# Autodesk Inventor assembly: aio_radiator_part
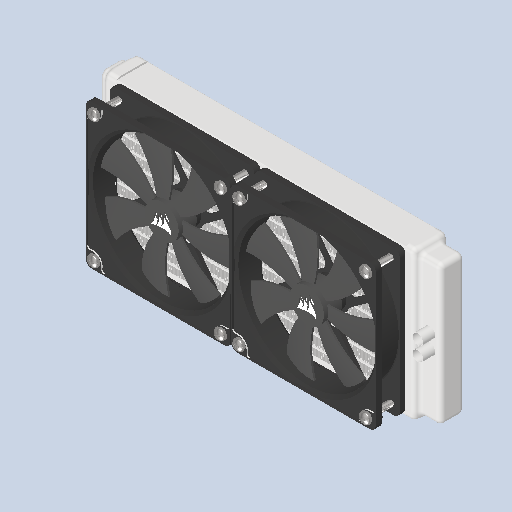
[picture p0: Inventor's stored thumbnail of the model, 512x512]
Saved by Autodesk Inventor 2022 (Build 260153000, 153)
## iProperties
Created: 2021-05-19
Part Number: aio_radiator_part
Document SubType Name: Assembly
Designer: 6128059
Author: 6128059
## Documents named in this file (9)
- C:\Users\sbbgi\Documents\GitHub\eatx_case\atx\resources\aio-cooler-1.snapshot.2\AIO Cooler\aio_radiator_part.iam
- C:\Users\sbbgi\Documents\GitHub\eatx_case\atx\resources\aio-cooler-1.snapshot.2\AIO Cooler\Kølerør.ipt
- C:\Users\sbbgi\Documents\GitHub\eatx_case\atx\resources\aio-cooler-1.snapshot.2\AIO Cooler\Gitter.ipt
- C:\Users\sbbgi\Documents\GitHub\eatx_case\atx\resources\aio-cooler-1.snapshot.2\AIO Cooler\Yderskal - Sheet metal.ipt
- C:\Users\sbbgi\Documents\GitHub\eatx_case\atx\resources\aio-cooler-1.snapshot.2\AIO Cooler\Radiator - Lukket ende.ipt
- C:\Users\sbbgi\Documents\GitHub\eatx_case\atx\resources\aio-cooler-1.snapshot.2\AIO Cooler\Radiator - Åben ende.ipt
- C:\Users\sbbgi\Documents\GitHub\eatx_case\atx\resources\aio-cooler-1.snapshot.2\AIO Cooler\120 mm fan assembly.iam
- C:\Users\sbbgi\Documents\GitHub\eatx_case\atx\resources\aio-cooler-1.snapshot.2\AIO Cooler\Rørende.ipt
- C:\Users\sbbgi\Documents\GitHub\eatx_case\atx\resources\aio-cooler-1.snapshot.2\AIO Cooler\ANSI B18.6.7M - M5x0,8 x 30(5).ipt
## Components (30 placed, 8 different names)
1. Kølerør:1 — Tangent:1, Mate:1, Tangent:2, Flush:1, Mate:11, Mate:12, Flush:2, Mate:13, Flush:3, Flush:4, Mate:14
2. Yderskal - Sheet metal:1 — Mate:8, Mate:9, Mate:10, Mate:11
3. Yderskal - Sheet metal:2 — Mate:2, Mate:3, Mate:4, Mate:5, Mate:6, Mate:7, Mate:12, Flush:2
4. 120 mm fan assembly:1 [sub-assembly] — Mate:2, Mate:3, Mate:4, Mate:10, Mate:32, Mate:33
5. 120 mm fan assembly:2 [sub-assembly] — Mate:5, Mate:6, Mate:7, Mate:8, Mate:9, Mate:30, Mate:31
6. Radiator - Åben ende:1 — Mate:13, Flush:3, Flush:4, Mate:15, Mate:16, Mate:20, Mate:21, Mate:22, Mate:23
7. Radiator - Lukket ende:1 — Mate:14, Mate:15, Mate:16
8. Rørende:3 — Mate:21, Mate:22
9. Rørende:4 — Mate:20, Mate:23
10. Gitter:1 — Tangent:1, Mate:1, Tangent:2, Flush:1
11. Gitter:2
12. Gitter:3
13. Gitter:4
14. Gitter:5
15. Gitter:6
16. Gitter:7
17. Gitter:8
18. Gitter:9
19. Gitter:10
20. Gitter:11
21. Gitter:12
22. Gitter:13
23. Cross Recessed Pan Head Machine Screw - Type IA - Metric M5x0,8 x 30:1 — Mate:30, Mate:31
24. Cross Recessed Pan Head Machine Screw - Type IA - Metric M5x0,8 x 30:2
25. Cross Recessed Pan Head Machine Screw - Type IA - Metric M5x0,8 x 30:3
26. Cross Recessed Pan Head Machine Screw - Type IA - Metric M5x0,8 x 30:4
27. Cross Recessed Pan Head Machine Screw - Type IA - Metric M5x0,8 x 30:5 — Mate:32, Mate:33
28. Cross Recessed Pan Head Machine Screw - Type IA - Metric M5x0,8 x 30:6
29. Cross Recessed Pan Head Machine Screw - Type IA - Metric M5x0,8 x 30:7
30. Cross Recessed Pan Head Machine Screw - Type IA - Metric M5x0,8 x 30:8
## Component patterns: (13 elements, first: Gitter:1), (4 elements, first: Cross Recessed Pan Head Machine Screw - Type IA - Metric M5x0,8 x 30:1), (4 elements, first: Cross Recessed Pan Head Machine Screw - Type IA - Metric M5x0,8 x 30:5)
## Relationships (30: Mate 24, Flush 4, Tangent 2)
- Tangent:1: Kølerør:1 ↔ Gitter:1
- Mate:1: Kølerør:1 ↔ Gitter:1
- Tangent:2: Kølerør:1 ↔ Gitter:1
- Flush:1: Kølerør:1 ↔ Gitter:1
- Mate:2: Yderskal - Sheet metal:2 ↔ 120 mm fan assembly:1
- Mate:3: Yderskal - Sheet metal:2 ↔ 120 mm fan assembly:1
- Mate:4: Yderskal - Sheet metal:2 ↔ 120 mm fan assembly:1
- Mate:5: Yderskal - Sheet metal:2 ↔ 120 mm fan assembly:2
- Mate:6: Yderskal - Sheet metal:2 ↔ 120 mm fan assembly:2
- Mate:7: Yderskal - Sheet metal:2 ↔ 120 mm fan assembly:2
- Mate:8: Yderskal - Sheet metal:1 ↔ 120 mm fan assembly:2
- Mate:9: Yderskal - Sheet metal:1 ↔ 120 mm fan assembly:2
- Mate:10: Yderskal - Sheet metal:1 ↔ 120 mm fan assembly:1
- Mate:11: Kølerør:1 ↔ Yderskal - Sheet metal:1
- Mate:12: Kølerør:1 ↔ Yderskal - Sheet metal:2
- Flush:2: Kølerør:1 ↔ Yderskal - Sheet metal:2
- Mate:13: Kølerør:1 ↔ Radiator - Åben ende:1
- Flush:3: Kølerør:1 ↔ Radiator - Åben ende:1
- Flush:4: Kølerør:1 ↔ Radiator - Åben ende:1
- Mate:14: Kølerør:1 ↔ Radiator - Lukket ende:1
- Mate:15: Radiator - Åben ende:1 ↔ Radiator - Lukket ende:1
- Mate:16: Radiator - Åben ende:1 ↔ Radiator - Lukket ende:1
- Mate:20: Radiator - Åben ende:1 ↔ Rørende:4
- Mate:21: Radiator - Åben ende:1 ↔ Rørende:3
- Mate:22 (5 mm): Radiator - Åben ende:1 ↔ Rørende:3
- Mate:23 (5 mm): Radiator - Åben ende:1 ↔ Rørende:4
- Mate:30: 120 mm fan assembly:2 ↔ Cross Recessed Pan Head Machine Screw - Type IA - Metric M5x0,8 x 30:1
- Mate:31: 120 mm fan assembly:2 ↔ Cross Recessed Pan Head Machine Screw - Type IA - Metric M5x0,8 x 30:1
- Mate:32: 120 mm fan assembly:1 ↔ Cross Recessed Pan Head Machine Screw - Type IA - Metric M5x0,8 x 30:5
- Mate:33: 120 mm fan assembly:1 ↔ Cross Recessed Pan Head Machine Screw - Type IA - Metric M5x0,8 x 30:5
